# Autodesk Inventor assembly: Fullenss sensor v3.1
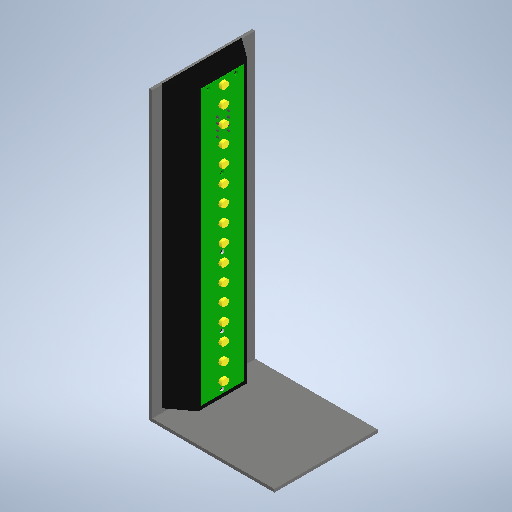
[picture p0: Inventor's stored thumbnail of the model, 512x512]
Saved by Autodesk Inventor 2025 (Build 290162000, 162)
## iProperties
Created: 2025-12-14
Part Number: Fullenss sensor v3.1
Document SubType Name: Assembly
Designer: kingc
Author: kingc
## Documents named in this file (4)
- C:\Users\kingc\OneDrive\Documents\Inventor Files\CSM\Fullenss sensor v3.1.iam
- C:\Users\kingc\OneDrive\Documents\Inventor Files\CSM\metal Back for v3.1.ipt
- C:\Users\kingc\OneDrive\Documents\Inventor Files\CSM\Fullenss sensor v3.1.ipt
- C:\Users\kingc\OneDrive\Documents\Inventor Files\CSM\Fullenss sensor v3.1 holder.ipt
## Components (3 placed, 3 different names)
1. metal Back for v3.1:1 — Mate:1, Mate:2, Mate:3
2. Fullenss sensor v3.1:1 — Mate:4, Mate:5, Mate:6
3. Fullenss sensor v3.1 holder:1 — Mate:1, Mate:2, Mate:3, Mate:4, Mate:5, Mate:6
## Relationships (6: Mate 6)
- Mate:1: metal Back for v3.1:1 ↔ Fullenss sensor v3.1 holder:1
- Mate:2: metal Back for v3.1:1 ↔ Fullenss sensor v3.1 holder:1
- Mate:3: metal Back for v3.1:1 ↔ Fullenss sensor v3.1 holder:1
- Mate:4: Fullenss sensor v3.1:1 ↔ Fullenss sensor v3.1 holder:1
- Mate:5: Fullenss sensor v3.1:1 ↔ Fullenss sensor v3.1 holder:1
- Mate:6: Fullenss sensor v3.1:1 ↔ Fullenss sensor v3.1 holder:1
